# Autodesk Inventor assembly: Lower box main assembly 2
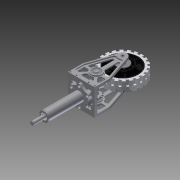
[picture p0: Inventor's stored thumbnail of the model, 180x180]
Saved by Autodesk Inventor 2012 (Build 160160000, 160)
## iProperties
Created: 2012-12-28
Part Number: Lower box main assembly 2
Document SubType Name: Assembly
Designer: Bryce
Author: Bryce
## Documents named in this file (14)
- C:\Users\Bryce\Dropbox\Inventor Design Project Files\Independent Swerves\Inventor 2012\Lower box main assembly 2.iam
- C:\Users\Bryce\Dropbox\Inventor Design Project Files\Independent Swerves\Inventor 2012\lower box upper plate.ipt
- C:\Users\Bryce\Dropbox\Inventor Design Project Files\Independent Swerves\Inventor 2012\lower bix side plate 2.ipt
- C:\Users\Bryce\Dropbox\Inventor Design Project Files\Independent Swerves\Inventor 2012\.375 ID .875 OD bearing.ipt
- C:\Users\Bryce\Dropbox\Inventor Design Project Files\Independent Swerves\Inventor 2012\lower box upper shaft.ipt
- C:\Users\Bryce\Dropbox\Inventor Design Project Files\Independent Swerves\Inventor 2012\lower box weel shaft steel.ipt
- C:\Users\Bryce\Dropbox\Inventor Design Project Files\Independent Swerves\Inventor 2012\lower box bolt plate.ipt
- C:\Users\Bryce\Dropbox\Inventor Design Project Files\Independent Swerves\Inventor 2012\.5 id 1.125 od flange bearing.ipt
- C:\Users\Bryce\Dropbox\Inventor Design Project Files\Independent Swerves\Inventor 2012\turn shaft 2.ipt
- C:\Users\Bryce\Dropbox\Inventor Design Project Files\Independent Swerves\Imported Components\miters.ipt
- C:\Users\Bryce\Dropbox\Inventor Design Project Files\Independent Swerves\Inventor 2012\vertical drive shaft 2.ipt
- C:\Users\Bryce\Dropbox\Inventor Design Project Files\Independent Swerves\Inventor 2012\wheel 4 in high grip.iam
- C:\Users\Bryce\Dropbox\Inventor Design Project Files\Independent Swerves\Imported Components\12t #25 sprocket.ipt
- C:\Users\Bryce\Dropbox\Inventor Design Project Files\Independent Swerves\Imported Components\36t #25 sprocket.ipt
## Components (16 placed, 13 different names)
1. lower box upper plate:1 — Mate:1, Mate:4, Mate:13, Mate:14, Mate:15, Mate:20, Mate:21, Mate:22, Mate:23
2. lower bix side plate 2:1 — Mate:1, Mate:7, Mate:12, Mate:20, Mate:21, Mate:25, Mate:49
3. lower bix side plate 2:2 — Mate:4, Mate:9, Mate:22, Mate:23, Mate:24, Flush:4, Mate:45
4. .375 ID .875 OD bearing:1 — Mate:7, Mate:11, Mate:25
5. .375 ID .875 OD bearing:2 — Mate:9, Mate:24
6. lower box upper shaft:1 — Mate:11, Mate:35, Flush:4, Mate:48, Rotation:1, Flush:7
7. lower box weel shaft steel:1 — Mate:12, Mate:27, Mate:28, Mate:43, Mate:49
8. lower box bolt plate:1 — Mate:13, Mate:14, Mate:15, Mate:18, Mate:26, Mate:50
9. turn shaft 2:1 — Mate:18, Mate:26, Mate:34, Mate:41, Mate:50
10. .5 id 1.125 od flange bearing:1 — Mate:27, Mate:42
11. .5 id 1.125 od flange bearing:2 — Mate:28, Mate:44
12. miters:1 — Mate:34, Mate:35, Flush:5
13. vertical drive shaft 2:1 — Mate:41, Flush:5, Rotation:1
14. wheel 4 in high grip:1 [sub-assembly] — Mate:42, Mate:43, Mate:44, Mate:45, Mate:54
15. 36t #25 sprocket:1 — Mate:54, Flush:9
16. 12t #25 sprocket:1 — Mate:48, Flush:7, Flush:9
## Relationships (38: Mate 32, Flush 4, RelateRotation 2)
- Mate:1: lower box upper plate:1 ↔ lower bix side plate 2:1
- Mate:4: lower box upper plate:1 ↔ lower bix side plate 2:2
- Mate:7: lower bix side plate 2:1 ↔ .375 ID .875 OD bearing:1
- Mate:9: lower bix side plate 2:2 ↔ .375 ID .875 OD bearing:2
- Mate:11: .375 ID .875 OD bearing:1 ↔ lower box upper shaft:1
- Mate:12: lower bix side plate 2:1 ↔ lower box weel shaft steel:1
- Mate:13: lower box upper plate:1 ↔ lower box bolt plate:1
- Mate:14: lower box upper plate:1 ↔ lower box bolt plate:1
- Mate:15: lower box upper plate:1 ↔ lower box bolt plate:1
- Mate:18: lower box bolt plate:1 ↔ turn shaft 2:1
- Mate:20: lower box upper plate:1 ↔ lower bix side plate 2:1
- Mate:21: lower box upper plate:1 ↔ lower bix side plate 2:1
- Mate:22: lower box upper plate:1 ↔ lower bix side plate 2:2
- Mate:23: lower box upper plate:1 ↔ lower bix side plate 2:2
- Mate:24: lower bix side plate 2:2 ↔ .375 ID .875 OD bearing:2
- Mate:25: lower bix side plate 2:1 ↔ .375 ID .875 OD bearing:1
- Mate:26: lower box bolt plate:1 ↔ turn shaft 2:1
- Mate:27: lower box weel shaft steel:1 ↔ .5 id 1.125 od flange bearing:1
- Mate:28: lower box weel shaft steel:1 ↔ .5 id 1.125 od flange bearing:2
- Mate:34: turn shaft 2:1 ↔ miters:1
- Mate:35: lower box upper shaft:1 ↔ miters:1
- Flush:4: lower bix side plate 2:2 ↔ lower box upper shaft:1
- Mate:41: turn shaft 2:1 ↔ vertical drive shaft 2:1
- Flush:5: miters:1 ↔ vertical drive shaft 2:1
- Mate:42: .5 id 1.125 od flange bearing:1 ↔ wheel 4 in high grip:1
- Mate:43: lower box weel shaft steel:1 ↔ wheel 4 in high grip:1
- Mate:44: .5 id 1.125 od flange bearing:2 ↔ wheel 4 in high grip:1
- Mate:45 (11.1125 mm): lower bix side plate 2:2 ↔ wheel 4 in high grip:1
- Mate:48: lower box upper shaft:1 ↔ 12t #25 sprocket:1
- Mate:49: lower bix side plate 2:1 ↔ lower box weel shaft steel:1
- Mate:50 (1.5875 mm): lower box bolt plate:1 ↔ turn shaft 2:1
- Rotation:1 [RelateRotation] (1 ul): lower box upper shaft:1 ↔ vertical drive shaft 2:1
- Flush:7: lower box upper shaft:1 ↔ 12t #25 sprocket:1
- [RelateRotation] (0.3333 ul): 36t #25 sprocket:1 ↔ 12t #25 sprocket:1
- [Mate]: wheel 4 in high grip:1 ↔ 36t #25 sprocket:1
- [Mate]: wheel 4 in high grip:1 ↔ 36t #25 sprocket:1
- Mate:54: wheel 4 in high grip:1 ↔ 36t #25 sprocket:1
- Flush:9: 36t #25 sprocket:1 ↔ 12t #25 sprocket:1
